# Autodesk Inventor assembly: 8dof_body
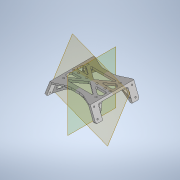
[picture p0: Inventor's stored thumbnail of the model, 180x180]
Saved by Autodesk Inventor 2020 (Build 240168000, 168)
## iProperties
Created: 2021-03-22
Part Number: 8dof_body
Document SubType Name: Assembly
Designer: Shuang Peng
Author: Shuang Peng
## Documents named in this file (2)
- D:\projects-3\biped_tiny\hardware\8dof_body.iam
- D:\projects-3\biped_tiny\hardware\body_linker_1_8d.ipt
## Components (1 placed, 1 different names)
1. body_linker_1_8d:1 — Flush:1, Flush:2
## Relationships (2: Flush 2)
- Flush:1: body_linker_1_8d:1
- Flush:2: body_linker_1_8d:1
